# Autodesk Inventor assembly: MOT_CIM-Motor_217-2000_MIR10
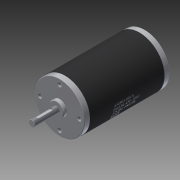
[picture p0: Inventor's stored thumbnail of the model, 180x180]
Saved by Autodesk Inventor 2016 SP1 (Build 200210100, 210)
## iProperties
Category: Motors
Company: Autodesk, Inc.
Created: 2015-12-10
Part Number: MOT_CIM-Motor_217-2000_MIR10
Project: FIRST
Catalog Web Link: http://www.vexrobotics.com/217-2000.html
Description: CIM Motor
Vendor: IFI
Document SubType Name: Assembly
Designer: steele
Mass: 972.526 g
Surface Area: 377.718 cm^2
Volume: 361.438 cm^3
Density: 2.69072 g/cm^3
Title: CIM Motor
Author: Autodesk, Inc.
## Documents named in this file (3)
- C:\snobotics\autodesk\2016\FRC KOP 2016\Motors\MOT_CIM-Motor_217-2000_MIR10.iam
- C:\snobotics\autodesk\2016\FRC KOP 2016\Motors\Parts\FR801-001_CIM Motor Body_MIR10.ipt
- C:\snobotics\autodesk\2016\FRC KOP 2016\Motors\Parts\FR801-001_CIM Motor Machine Screw_MIR10.ipt
## Components (3 placed, 2 different names)
1. FR801-001_CIM Motor Body_MIR10:1 — Insert:1, Insert:2
2. FR801-001_CIM Motor Machine Screw_MIR10:1 — Insert:1
3. FR801-001_CIM Motor Machine Screw_MIR10:2 — Insert:2
## Relationships (2: Insert 2)
- Insert:1: FR801-001_CIM Motor Body_MIR10:1 ↔ FR801-001_CIM Motor Machine Screw_MIR10:1
- Insert:2: FR801-001_CIM Motor Body_MIR10:1 ↔ FR801-001_CIM Motor Machine Screw_MIR10:2
